# Autodesk Inventor assembly: 右後脚ユニット4
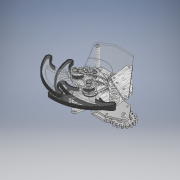
[picture p0: Inventor's stored thumbnail of the model, 180x180]
Saved by Autodesk Inventor 2020 (Build 240168000, 168)
## iProperties
Created: 2019-08-30
Part Number: 右後脚ユニット4
Document SubType Name: Assembly
Designer: 雪村
Mass: 248.848 g
Surface Area: 1222.45 cm^2
Volume: 119.079 cm^3
Density: 2.08977 g/cm^3
Author: 雪村
## Documents named in this file (14)
- C:\Users\white\Documents\SRDC\SRDC\Inventor_2017\2018年機体\2020年4年機体\右後脚ユニット4.iam
- C:\Users\white\Documents\SRDC\SRDC\Inventor_2017\2018年機体\2020年4年機体\脚クランク1.iam
- C:\Users\white\Documents\SRDC\SRDC\Inventor_2017\2018年機体\2020年4年機体\脚最終段カム1.ipt
- C:\Users\white\Documents\SRDC\SRDC\Inventor_2017\2018年機体\パーツ\オイレスフランジ付き12142006.ipt
- C:\Users\white\Documents\SRDC\SRDC\Inventor_2017\2018年機体\パーツ\スペーサーm3,35.ipt
- C:\Users\white\Documents\SRDC\SRDC\Inventor_2017\2018年機体\2020年4年機体\歯車m2.z21.2.ipt
- C:\Users\white\Documents\SRDC\SRDC\Inventor_2017\2018年機体\2020年4年機体\脚最終段抑え1.ipt
- C:\Users\white\Documents\SRDC\SRDC\Inventor_2017\2018年機体\パーツ\スペーサーm3,11.ipt
- C:\Users\white\Documents\SRDC\SRDC\Inventor_2017\2018年機体\2020年4年機体\後脚ユニット締結パーツ4_MIR.ipt
- C:\Users\white\Documents\SRDC\SRDC\Inventor_2017\2018年機体\2020年4年機体\後脚ギアトレイン3_MIR.iam
- C:\Users\white\Documents\SRDC\SRDC\Inventor_2017\2018年機体\2020年4年機体\脚内フレーム4.ipt
- C:\Users\white\Documents\SRDC\SRDC\Inventor_2017\2018年機体\2020年4年機体\ヘッケン＋揺動節1_MIR.iam
- C:\Users\white\Documents\SRDC\SRDC\Inventor_2017\2018年機体\2020年4年機体\脚外フレーム3.ipt
- C:\Users\white\Documents\SRDC\SRDC\Inventor_2017\2018年機体\2020年4年機体\脚最終段カム2.ipt
## Components (21 placed, 13 different names)
1. 脚内フレーム4:1 — 挿入:26
2. 脚クランク1:1 [sub-assembly]
3. オイレスフランジ付き12142006:1
4. スペーサーm3,35:1
5. スペーサーm3,35:2
6. ヘッケン＋揺動節1_MIR:1 [sub-assembly]
7. ヘッケン＋揺動節1_MIR:2 [sub-assembly]
8. ヘッケン＋揺動節1_MIR:3 [sub-assembly]
9. ヘッケン＋揺動節1_MIR:4 [sub-assembly]
10. スペーサーm3,35:3
11. 脚最終段カム1:1
12. 歯車m2.z21.2:1
13. 脚外フレーム3:1 — 挿入:24, 挿入:25
14. 脚最終段抑え1:1
15. スペーサーm3,11:1
16. スペーサーm3,11:2
17. スペーサーm3,11:3
18. 脚最終段カム2:1
19. オイレスフランジ付き12142006:2
20. 後脚ユニット締結パーツ4_MIR:1 — 挿入:24, 挿入:25, メイト:5
21. 後脚ギアトレイン3_MIR:1 [sub-assembly] — 挿入:26, メイト:5
## Relationships (31: Insert 26, Mate 5)
- [Insert]: 脚クランク1:1 ↔ ヘッケン＋揺動節1_MIR:1
- [Insert]: 脚クランク1:1 ↔ ヘッケン＋揺動節1_MIR:2
- [Insert]: 脚クランク1:1 ↔ ヘッケン＋揺動節1_MIR:4
- [Insert]: 脚クランク1:1 ↔ ヘッケン＋揺動節1_MIR:3
- [Mate]: スペーサーm3,35:1 ↔ ヘッケン＋揺動節1_MIR:3
- [Mate]: スペーサーm3,35:1 ↔ ヘッケン＋揺動節1_MIR:4
- [Mate]: スペーサーm3,35:1 ↔ ヘッケン＋揺動節1_MIR:1
- [Mate]: スペーサーm3,35:1 ↔ ヘッケン＋揺動節1_MIR:2
- [Insert]: 脚クランク1:1 ↔ 脚最終段カム1:1
- [Insert]: 脚クランク1:1 ↔ 脚最終段カム1:1
- [Insert]: オイレスフランジ付き12142006:1 ↔ 脚最終段カム1:1
- [Insert]: 脚最終段カム1:1 ↔ 歯車m2.z21.2:1
- [Insert]: 脚最終段カム1:1 ↔ 歯車m2.z21.2:1
- [Insert]: 脚内フレーム4:1 ↔ スペーサーm3,35:1
- [Insert]: 脚内フレーム4:1 ↔ オイレスフランジ付き12142006:1
- [Insert]: 脚内フレーム4:1 ↔ スペーサーm3,35:3
- [Insert]: 脚内フレーム4:1 ↔ スペーサーm3,35:2
- [Insert]: スペーサーm3,35:1 ↔ 脚外フレーム3:1
- [Insert]: スペーサーm3,35:3 ↔ 脚外フレーム3:1
- [Insert]: 脚内フレーム4:1 ↔ スペーサーm3,11:1
- [Insert]: 脚内フレーム4:1 ↔ スペーサーm3,11:2
- [Insert]: 脚内フレーム4:1 ↔ スペーサーm3,11:3
- [Insert]: 脚最終段抑え1:1 ↔ スペーサーm3,11:2
- [Insert]: 脚最終段抑え1:1 ↔ スペーサーm3,11:1
- [Insert]: 歯車m2.z21.2:1 ↔ 脚最終段カム2:1
- [Insert]: 歯車m2.z21.2:1 ↔ 脚最終段カム2:1
- [Insert]: 脚最終段カム2:1 ↔ オイレスフランジ付き12142006:2
- 挿入:24 [Insert]: 脚外フレーム3:1 ↔ 後脚ユニット締結パーツ4_MIR:1
- 挿入:25 [Insert]: 脚外フレーム3:1 ↔ 後脚ユニット締結パーツ4_MIR:1
- 挿入:26 [Insert]: 脚内フレーム4:1 ↔ 後脚ギアトレイン3_MIR:1
- メイト:5 [Mate]: 後脚ユニット締結パーツ4_MIR:1 ↔ 後脚ギアトレイン3_MIR:1
## Named parameters: d28_d35 = 0 mm, d36_d44 = 0 mm, d37_d45 = 0 mm, d10_d12 = 0 mm
